# Autodesk Inventor assembly: 関節2
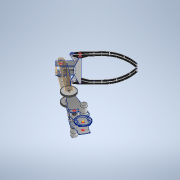
[picture p0: Inventor's stored thumbnail of the model, 180x180]
Saved by Autodesk Inventor 2021 (Build 250183000, 183)
## iProperties
Created: 2022-02-02
Part Number: 関節2
Document SubType Name: Assembly
Designer: hirohumi
Mass: 2155.98 g
Surface Area: 6804.47 cm^2
Volume: 1355.22 cm^3
Density: 1.59087 g/cm^3
Author: hirohumi
## Documents named in this file (8)
- C:\Users\hirohumi\OneDrive\ドキュメント\ロボ研\2022NHKロボコン\R2_version1\3軸アームver2\関節2.iam
- C:\Users\hirohumi\OneDrive\ドキュメント\ロボ研\2022NHKロボコン\R2_version1\3軸アーム\軸8-80.ipt
- C:\Users\hirohumi\OneDrive\ドキュメント\ロボ研\2022NHKロボコン\R2_version1\3軸アームver2\関節2_側板.ipt
- C:\Users\hirohumi\OneDrive\ドキュメント\ロボ研\2022NHKロボコン\R2_version1\3軸アーム\プーリ_歯数60.ipt
- C:\Users\hirohumi\OneDrive\ドキュメント\ロボ研\2022NHKロボコン\R2_version1\R2_ハンド.iam
- C:\Users\hirohumi\OneDrive\ドキュメント\ロボ研\2022NHKロボコン\R2_version1\3軸アーム\関節1_プーリ2個.iam
- C:\Users\hirohumi\OneDrive\ドキュメント\ロボ研\2022NHKロボコン\R2_version1\3軸アームver2\関節3.iam
- C:\Users\hirohumi\OneDrive\ドキュメント\ロボ研\2022NHKロボコン\R2_version1\3軸アームver2\関節2_上板.ipt
## Components (12 placed, 7 different names)
1. 軸8-80:1 — 挿入:1, 挿入:3
2. 軸8-80:2 — 挿入:2, 挿入:4
3. 関節2_側板:1 — 挿入:1, 挿入:2, 挿入:7, 挿入:8
4. 関節2_側板:2 — 挿入:3, 挿入:4, 挿入:9, 挿入:10, 挿入:11, 挿入:12
5. プーリ_歯数60:1 — 挿入:5, 挿入:6, メイト:6
6. プーリ_歯数60:2 — 挿入:5, 挿入:6, 挿入:7, 挿入:8
7. 軸8-80:3 — 挿入:10, メイト:3, メイト:4
8. 軸8-80:4 — 挿入:9, メイト:1
9. R2_ハンド:1 [sub-assembly] — メイト:1, フラッシュ:1
10. 関節3:1 [sub-assembly] — メイト:3, メイト:5, メイト:6
11. 関節1_プーリ2個:1 [sub-assembly] — メイト:4, メイト:5, フラッシュ:1
12. 関節2_上板:1 — 挿入:11, 挿入:12
## Relationships (18: Insert 12, Mate 5, Flush 1)
- 挿入:1 [Insert]: 軸8-80:1 ↔ 関節2_側板:1
- 挿入:2 [Insert]: 軸8-80:2 ↔ 関節2_側板:1
- 挿入:3 [Insert]: 軸8-80:1 ↔ 関節2_側板:2
- 挿入:4 [Insert]: 軸8-80:2 ↔ 関節2_側板:2
- 挿入:5 [Insert]: プーリ_歯数60:1 ↔ プーリ_歯数60:2
- 挿入:6 [Insert]: プーリ_歯数60:1 ↔ プーリ_歯数60:2
- 挿入:7 [Insert]: 関節2_側板:1 ↔ プーリ_歯数60:2
- 挿入:8 [Insert]: 関節2_側板:1 ↔ プーリ_歯数60:2
- 挿入:9 [Insert]: 関節2_側板:2 ↔ 軸8-80:4
- 挿入:10 [Insert]: 関節2_側板:2 ↔ 軸8-80:3
- メイト:1 [Mate]: 軸8-80:4 ↔ R2_ハンド:1
- メイト:3 [Mate]: 軸8-80:3 ↔ 関節3:1
- メイト:4 [Mate]: 軸8-80:3 ↔ 関節1_プーリ2個:1
- メイト:5 [Mate]: 関節3:1 ↔ 関節1_プーリ2個:1
- 挿入:11 [Insert]: 関節2_側板:2 ↔ 関節2_上板:1
- 挿入:12 [Insert]: 関節2_側板:2 ↔ 関節2_上板:1
- メイト:6 [Mate]: プーリ_歯数60:1 ↔ 関節3:1
- フラッシュ:1 [Flush]: R2_ハンド:1 ↔ 関節1_プーリ2個:1
